# Autodesk Inventor assembly: Roller Assembled
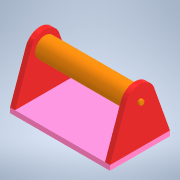
[picture p0: Inventor's stored thumbnail of the model, 180x180]
Saved by Autodesk Inventor 2022.4 (Build 264492000, 492)
## iProperties
Created: 2024-02-15
Part Number: Roller Assembled
Document SubType Name: Assembly
Designer: t60147996
Author: t60147996
## Documents named in this file (4)
- D:\Spring 2024\Advanced CAD\Roller Assembled.iam
- D:\Spring 2024\Advanced CAD\Roller Frame.ipt
- D:\Spring 2024\Advanced CAD\Roller Base.ipt
- D:\Spring 2024\Advanced CAD\Roller Pin.ipt
## Components (4 placed, 3 different names)
1. Roller Frame:1 — Mate:5, Flush:1, Mate:7
2. Roller Frame:2 — Mate:1, Mate:3, Mate:6, Flush:2, Mate:8, Mate:9
3. Roller Base:1 — Mate:1, Mate:3, Mate:5, Mate:6, Flush:1, Flush:2
4. Roller Pin:1 — Mate:7, Mate:8, Mate:9
## Relationships (9: Mate 7, Flush 2)
- Mate:1: Roller Frame:2 ↔ Roller Base:1
- Mate:3: Roller Frame:2 ↔ Roller Base:1
- Mate:5: Roller Frame:1 ↔ Roller Base:1
- Mate:6: Roller Frame:2 ↔ Roller Base:1
- Flush:1: Roller Frame:1 ↔ Roller Base:1
- Flush:2: Roller Frame:2 ↔ Roller Base:1
- Mate:7: Roller Frame:1 ↔ Roller Pin:1
- Mate:8: Roller Frame:2 ↔ Roller Pin:1
- Mate:9: Roller Frame:2 ↔ Roller Pin:1
